# Autodesk Inventor assembly: Linear Actuator
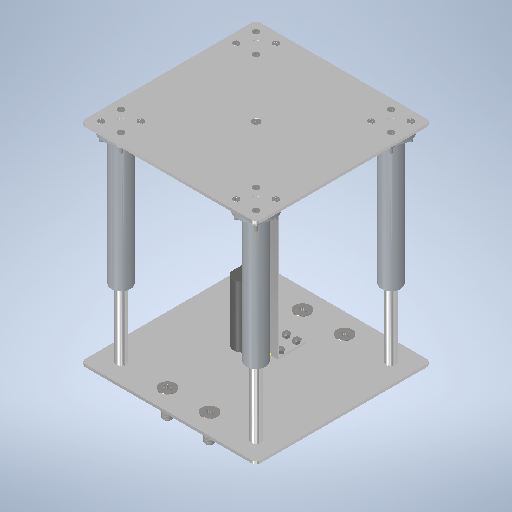
[picture p0: Inventor's stored thumbnail of the model, 512x512]
Saved by Autodesk Inventor 2025 (Build 290162000, 162)
## iProperties
Created: 2025-10-15
Part Number: Linear Actuator
Document SubType Name: Assembly
Designer: Haggag
Author: Haggag
## Documents named in this file (19)
- D:\gp amr\Lifting Mechanism 150mm\Lifting Mechanism 150mm\Linear Actuator.iam
- D:\gp amr\Lifting Mechanism 150mm\Lifting Mechanism 150mm\Actuonix-P16-150-256-12-P-Housing.ipt
- D:\gp amr\Lifting Mechanism 150mm\Lifting Mechanism 150mm\Actuonix-P16-150-256-12-P-Shaft.ipt
- D:\gp amr\Lifting Mechanism 150mm\Lifting Mechanism 150mm\Base.ipt
- D:\gp amr\Lifting Mechanism 150mm\Lifting Mechanism 150mm\Linear Actuator Base Holder.ipt
- D:\gp amr\Lifting Mechanism 150mm\Lifting Mechanism 150mm\Linear Actuator Plate Holder.ipt
- D:\gp amr\Lifting Mechanism 150mm\Lifting Mechanism 150mm\Plate.ipt
- D:\gp amr\Lifting Mechanism 150mm\Lifting Mechanism 150mm\Bracket Holder.ipt
- D:\gp amr\Lifting Mechanism 150mm\Lifting Mechanism 150mm\Bracket.ipt
- D:\gp amr\Lifting Mechanism 150mm\Lifting Mechanism 150mm\Plate Support.ipt
- D:\gp amr\Lifting Mechanism 150mm\Lifting Mechanism 150mm\LMEF12LUU.ipt
- C:\Users\hp\OneDrive - Faculty of Engineering Ain Shams University\Documents\Inventor\Content Center Files\R2025\en-US\AS 1427(07)\AS 1427 - M5 x 12(6) II.ipt
- C:\Users\hp\OneDrive - Faculty of Engineering Ain Shams University\Documents\Inventor\Content Center Files\R2025\en-US\AS 1427(04)\AS 1427 - M4 x 10(5) I.ipt
- C:\Users\hp\OneDrive - Faculty of Engineering Ain Shams University\Documents\Inventor\Content Center Files\R2025\en-US\AS 1112 (2)\AS 1112 - M4  Type 5.ipt
- C:\Users\hp\OneDrive - Faculty of Engineering Ain Shams University\Documents\Inventor\Content Center Files\R2025\en-US\AS 1427(04)\AS 1427 - M4 x 20(5) I.ipt
- C:\Users\hp\OneDrive - Faculty of Engineering Ain Shams University\Documents\Inventor\Content Center Files\R2025\en-US\AS 1427(04)\AS 1427 - M2 x 8(5) I.ipt
- C:\Users\hp\OneDrive - Faculty of Engineering Ain Shams University\Documents\Inventor\Content Center Files\R2025\en-US\BS 3692(1)\BS 3692 - M2(1).ipt
- C:\Users\hp\OneDrive - Faculty of Engineering Ain Shams University\Documents\Inventor\Content Center Files\R2025\en-US\AS 1112 (2)\AS 1112 - M2  Type 5.ipt
- C:\Users\hp\OneDrive - Faculty of Engineering Ain Shams University\Documents\Inventor\Content Center Files\R2025\en-US\AS 1427(07)\AS 1427 - M10 x 30(6) II.ipt
## Components (76 placed, 18 different names)
1. Actuonix-P16-150-256-12-P-Housing:1 — Cylindrical:1, Rotational:2, Angle:1, Slider:1
2. Actuonix-P16-150-256-12-P-Shaft:1 — Cylindrical:1, Rigid:2
3. Base:2 — Rigid:1, Rigid:15, Rigid:34, Rigid:35, Rigid:36, Rigid:37, Rigid:73, Rigid:74, Rigid:75, Rigid:76, Rigid:77, Flush:1, Rigid:78, Rigid:79, Rigid:80, Rigid:81
4. Linear Actuator Base Holder:1 — Rotational:2, Rigid:1, Rigid:24, Rigid:38
5. Linear Actuator Plate Holder:1 — Rigid:2, Rotational:5, Rigid:39, Rigid:40
6. Plate:1 — Rotational:5, Rigid:10, Rigid:13, Rigid:11, Rigid:12, Rigid:14, Rigid:42, Rigid:43, Rigid:44, Rigid:45, Rotational:9, Rigid:50, Rigid:51, Rigid:52, Rigid:53, Rigid:54, Rigid:55, Rigid:56, Rigid:57, Rigid:58, Rigid:59, Rigid:60
7. Bracket Holder:1 — Rigid:3, Rigid:21, Rigid:20, Rigid:22, Rigid:23, Rigid:30, Rigid:31, Rigid:32, Rigid:33
8. Bracket:1 — Angle:1, Slider:1, Rigid:3, Insert:1, Rigid:26, Rigid:27, Rigid:28, Rigid:29, Rigid:41
9. Plate Support:1 — Rigid:74, Rigid:77
10. Plate Support:2 — Rigid:73
11. Plate Support:3 — Rigid:75
12. Plate Support:4 — Rigid:76
13. LMEF12LUU:1 — Rigid:11, Rigid:65, Rigid:66, Rigid:67, Rigid:68
14. LMEF12LUU:2 — Rigid:12, Rigid:61, Rigid:62, Rigid:63, Rigid:64
15. LMEF12LUU:3 — Rigid:13, Rigid:69, Rigid:70, Rigid:71, Rigid:72
16. LMEF12LUU:4 — Rigid:10, Rigid:46, Rigid:47, Rigid:48, Rigid:49
17. AS 1427 Z - Metric M5 x 12:1 — Rigid:14
18. AS 1427 Z - Metric M5 x 12:2 — Rigid:15, Flush:1
19. AS 1112 (2) - Metric M4  Type 5:1 — Rigid:21
20. AS 1112 (2) - Metric M4  Type 5:2 — Rigid:22
21. AS 1112 (2) - Metric M4  Type 5:3 — Rigid:20
22. AS 1112 (2) - Metric M4  Type 5:4 — Rigid:23
23. AS 1112 (2) - Metric M4  Type 5:5 — Rigid:24
24. BS 3692 - Metric M2:1 — Insert:1
25. AS 1427 H - Metric M2 x 8:2 — Rigid:28
26. AS 1427 H - Metric M2 x 8:3 — Rigid:29
27. AS 1427 H - Metric M2 x 8:4 — Rigid:26
28. AS 1427 H - Metric M2 x 8:5 — Rigid:27
29. AS 1112 (2) - Metric M2  Type 5:1 — Rigid:30
30. AS 1112 (2) - Metric M2  Type 5:2 — Rigid:33
31. AS 1112 (2) - Metric M2  Type 5:3 — Rigid:31
32. AS 1112 (2) - Metric M2  Type 5:4 — Rigid:32
33. AS 1427 H - Metric M4 x 10:5 — Rigid:34
34. AS 1427 H - Metric M4 x 10:6 — Rigid:36
35. AS 1427 H - Metric M4 x 10:7 — Rigid:35
36. AS 1427 H - Metric M4 x 10:8 — Rigid:37
37. AS 1427 H - Metric M4 x 20:1 — Rigid:38
38. AS 1427 H - Metric M4 x 20:2 — Rigid:39
39. AS 1112 (2) - Metric M4  Type 5:7 — Rigid:40
40. AS 1427 H - Metric M2 x 8:6 — Rigid:41
41. AS 1427 H - Metric M4 x 20:3 — Rigid:42
42. AS 1427 H - Metric M4 x 20:4 — Rigid:43
43. AS 1427 H - Metric M4 x 20:5 — Rigid:44
44. AS 1427 H - Metric M4 x 20:6 — Rigid:45
45. AS 1112 (2) - Metric M4  Type 5:8 — Rigid:46
46. AS 1112 (2) - Metric M4  Type 5:9 — Rigid:47
47. AS 1112 (2) - Metric M4  Type 5:10 — Rigid:49
48. AS 1112 (2) - Metric M4  Type 5:11 — Rigid:48
49. AS 1427 H - Metric M4 x 20:7 — Rigid:50
50. AS 1427 H - Metric M4 x 20:8 — Rigid:52
51. AS 1427 H - Metric M4 x 20:9 — Rigid:51
52. AS 1427 H - Metric M4 x 20:10 — Rotational:9
53. AS 1427 H - Metric M4 x 20:11 — Rigid:56
54. AS 1427 H - Metric M4 x 20:12 — Rigid:55
55. AS 1427 H - Metric M4 x 20:14 — Rigid:53
56. AS 1427 H - Metric M4 x 20:15 — Rigid:54
57. AS 1427 H - Metric M4 x 20:16 — Rigid:59
58. AS 1427 H - Metric M4 x 20:17 — Rigid:58
59. AS 1427 H - Metric M4 x 20:18 — Rigid:57
60. AS 1427 H - Metric M4 x 20:19 — Rigid:60
61. AS 1112 (2) - Metric M4  Type 5:12 — Rigid:61
62. AS 1112 (2) - Metric M4  Type 5:13 — Rigid:64
63. AS 1112 (2) - Metric M4  Type 5:14 — Rigid:62
64. AS 1112 (2) - Metric M4  Type 5:15 — Rigid:63
65. AS 1112 (2) - Metric M4  Type 5:16 — Rigid:65
66. AS 1427 Z - Metric M10 x 30:2 — Rigid:79
67. AS 1112 (2) - Metric M4  Type 5:17 — Rigid:66
68. AS 1112 (2) - Metric M4  Type 5:18 — Rigid:67
69. AS 1427 Z - Metric M10 x 30:3 — Rigid:80
70. AS 1112 (2) - Metric M4  Type 5:19 — Rigid:68
71. AS 1112 (2) - Metric M4  Type 5:20 — Rigid:69
72. AS 1427 Z - Metric M10 x 30:4 — Rigid:81
73. AS 1112 (2) - Metric M4  Type 5:21 — Rigid:72
74. AS 1112 (2) - Metric M4  Type 5:22 — Rigid:71
75. AS 1112 (2) - Metric M4  Type 5:23 — Rigid:70
76. AS 1427 Z - Metric M10 x 30:1 — Rigid:78
## Relationships (78: WeldJoint 70, RevoluteJoint 3, CylindricalJoint 1, Angle 1, TranslationJoint 1, Insert 1, Flush 1)
- Cylindrical:1: Actuonix-P16-150-256-12-P-Housing:1 ↔ Actuonix-P16-150-256-12-P-Shaft:1
- Rotational:2 [RevoluteJoint]: Actuonix-P16-150-256-12-P-Housing:1 ↔ Linear Actuator Base Holder:1
- Rigid:1 [WeldJoint]: Base:2 ↔ Linear Actuator Base Holder:1
- Rigid:2 [WeldJoint] (-0.7 mm): Actuonix-P16-150-256-12-P-Shaft:1 ↔ Linear Actuator Plate Holder:1
- Rotational:5 [RevoluteJoint]: Linear Actuator Plate Holder:1 ↔ Plate:1
- Angle:1 (0 deg): Actuonix-P16-150-256-12-P-Housing:1 ↔ Bracket:1
- Slider:1 [TranslationJoint]: Actuonix-P16-150-256-12-P-Housing:1 ↔ Bracket:1
- Rigid:3 [WeldJoint]: Bracket Holder:1 ↔ Bracket:1
- Rigid:10 [WeldJoint]: Plate:1 ↔ LMEF12LUU:4
- Rigid:13 [WeldJoint]: Plate:1 ↔ LMEF12LUU:3
- Rigid:11 [WeldJoint]: Plate:1 ↔ LMEF12LUU:1
- Rigid:12 [WeldJoint]: Plate:1 ↔ LMEF12LUU:2
- Rigid:15 [WeldJoint]: Base:2 ↔ AS 1427 Z - Metric M5 x 12:2
- Rigid:14 [WeldJoint]: Plate:1 ↔ AS 1427 Z - Metric M5 x 12:1
- Rigid:21 [WeldJoint]: Bracket Holder:1 ↔ AS 1112 (2) - Metric M4  Type 5:1
- Rigid:20 [WeldJoint]: Bracket Holder:1 ↔ AS 1112 (2) - Metric M4  Type 5:3
- Rigid:22 [WeldJoint]: Bracket Holder:1 ↔ AS 1112 (2) - Metric M4  Type 5:2
- Rigid:23 [WeldJoint]: Bracket Holder:1 ↔ AS 1112 (2) - Metric M4  Type 5:4
- Rigid:24 [WeldJoint]: Linear Actuator Base Holder:1 ↔ AS 1112 (2) - Metric M4  Type 5:5
- Insert:1: Bracket:1 ↔ BS 3692 - Metric M2:1
- Rigid:26 [WeldJoint]: Bracket:1 ↔ AS 1427 H - Metric M2 x 8:4
- Rigid:27 [WeldJoint]: Bracket:1 ↔ AS 1427 H - Metric M2 x 8:5
- Rigid:28 [WeldJoint]: Bracket:1 ↔ AS 1427 H - Metric M2 x 8:2
- Rigid:29 [WeldJoint]: Bracket:1 ↔ AS 1427 H - Metric M2 x 8:3
- Rigid:30 [WeldJoint]: Bracket Holder:1 ↔ AS 1112 (2) - Metric M2  Type 5:1
- Rigid:31 [WeldJoint]: Bracket Holder:1 ↔ AS 1112 (2) - Metric M2  Type 5:3
- Rigid:32 [WeldJoint]: Bracket Holder:1 ↔ AS 1112 (2) - Metric M2  Type 5:4
- Rigid:33 [WeldJoint]: Bracket Holder:1 ↔ AS 1112 (2) - Metric M2  Type 5:2
- Rigid:34 [WeldJoint]: Base:2 ↔ AS 1427 H - Metric M4 x 10:5
- Rigid:35 [WeldJoint]: Base:2 ↔ AS 1427 H - Metric M4 x 10:7
- Rigid:36 [WeldJoint]: Base:2 ↔ AS 1427 H - Metric M4 x 10:6
- Rigid:37 [WeldJoint]: Base:2 ↔ AS 1427 H - Metric M4 x 10:8
- Rigid:38 [WeldJoint]: Linear Actuator Base Holder:1 ↔ AS 1427 H - Metric M4 x 20:1
- Rigid:39 [WeldJoint]: Linear Actuator Plate Holder:1 ↔ AS 1427 H - Metric M4 x 20:2
- Rigid:40 [WeldJoint]: Linear Actuator Plate Holder:1 ↔ AS 1112 (2) - Metric M4  Type 5:7
- Rigid:41 [WeldJoint]: Bracket:1 ↔ AS 1427 H - Metric M2 x 8:6
- Rigid:42 [WeldJoint]: Plate:1 ↔ AS 1427 H - Metric M4 x 20:3
- Rigid:43 [WeldJoint]: Plate:1 ↔ AS 1427 H - Metric M4 x 20:4
- Rigid:44 [WeldJoint]: Plate:1 ↔ AS 1427 H - Metric M4 x 20:5
- Rigid:45 [WeldJoint]: Plate:1 ↔ AS 1427 H - Metric M4 x 20:6
- Rigid:46 [WeldJoint]: LMEF12LUU:4 ↔ AS 1112 (2) - Metric M4  Type 5:8
- Rigid:47 [WeldJoint]: LMEF12LUU:4 ↔ AS 1112 (2) - Metric M4  Type 5:9
- Rigid:48 [WeldJoint]: LMEF12LUU:4 ↔ AS 1112 (2) - Metric M4  Type 5:11
- Rigid:49 [WeldJoint]: LMEF12LUU:4 ↔ AS 1112 (2) - Metric M4  Type 5:10
- Rotational:9 [RevoluteJoint]: Plate:1 ↔ AS 1427 H - Metric M4 x 20:10
- Rigid:50 [WeldJoint]: Plate:1 ↔ AS 1427 H - Metric M4 x 20:7
- Rigid:51 [WeldJoint]: Plate:1 ↔ AS 1427 H - Metric M4 x 20:9
- Rigid:52 [WeldJoint]: Plate:1 ↔ AS 1427 H - Metric M4 x 20:8
- Rigid:53 [WeldJoint]: Plate:1 ↔ AS 1427 H - Metric M4 x 20:14
- Rigid:54 [WeldJoint]: Plate:1 ↔ AS 1427 H - Metric M4 x 20:15
- Rigid:55 [WeldJoint]: Plate:1 ↔ AS 1427 H - Metric M4 x 20:12
- Rigid:56 [WeldJoint]: Plate:1 ↔ AS 1427 H - Metric M4 x 20:11
- Rigid:57 [WeldJoint]: Plate:1 ↔ AS 1427 H - Metric M4 x 20:18
- Rigid:58 [WeldJoint]: Plate:1 ↔ AS 1427 H - Metric M4 x 20:17
- Rigid:59 [WeldJoint]: Plate:1 ↔ AS 1427 H - Metric M4 x 20:16
- Rigid:60 [WeldJoint]: Plate:1 ↔ AS 1427 H - Metric M4 x 20:19
- Rigid:61 [WeldJoint]: LMEF12LUU:2 ↔ AS 1112 (2) - Metric M4  Type 5:12
- Rigid:62 [WeldJoint]: LMEF12LUU:2 ↔ AS 1112 (2) - Metric M4  Type 5:14
- Rigid:63 [WeldJoint]: LMEF12LUU:2 ↔ AS 1112 (2) - Metric M4  Type 5:15
- Rigid:64 [WeldJoint]: LMEF12LUU:2 ↔ AS 1112 (2) - Metric M4  Type 5:13
- Rigid:65 [WeldJoint]: LMEF12LUU:1 ↔ AS 1112 (2) - Metric M4  Type 5:16
- Rigid:66 [WeldJoint]: LMEF12LUU:1 ↔ AS 1112 (2) - Metric M4  Type 5:17
- Rigid:67 [WeldJoint]: LMEF12LUU:1 ↔ AS 1112 (2) - Metric M4  Type 5:18
- Rigid:68 [WeldJoint]: LMEF12LUU:1 ↔ AS 1112 (2) - Metric M4  Type 5:19
- Rigid:69 [WeldJoint]: LMEF12LUU:3 ↔ AS 1112 (2) - Metric M4  Type 5:20
- Rigid:70 [WeldJoint]: LMEF12LUU:3 ↔ AS 1112 (2) - Metric M4  Type 5:23
- Rigid:71 [WeldJoint]: LMEF12LUU:3 ↔ AS 1112 (2) - Metric M4  Type 5:22
- Rigid:72 [WeldJoint]: LMEF12LUU:3 ↔ AS 1112 (2) - Metric M4  Type 5:21
- Rigid:73 [WeldJoint]: Base:2 ↔ Plate Support:2
- Rigid:74 [WeldJoint]: Base:2 ↔ Plate Support:1
- Rigid:75 [WeldJoint]: Base:2 ↔ Plate Support:3
- Rigid:76 [WeldJoint]: Base:2 ↔ Plate Support:4
- Rigid:77 [WeldJoint]: Base:2 ↔ Plate Support:1
- Flush:1: Base:2 ↔ AS 1427 Z - Metric M5 x 12:2
- Rigid:78 [WeldJoint]: Base:2 ↔ AS 1427 Z - Metric M10 x 30:1
- Rigid:79 [WeldJoint]: Base:2 ↔ AS 1427 Z - Metric M10 x 30:2
- Rigid:80 [WeldJoint]: Base:2 ↔ AS 1427 Z - Metric M10 x 30:3
- Rigid:81 [WeldJoint]: Base:2 ↔ AS 1427 Z - Metric M10 x 30:4
